# Autodesk Inventor assembly: L3 Gearbox Assembly
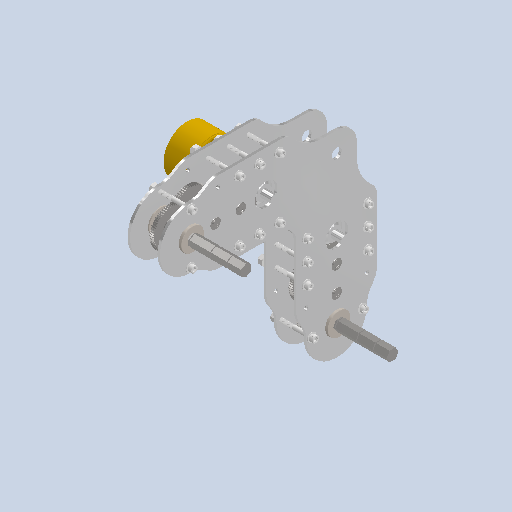
[picture p0: Inventor's stored thumbnail of the model, 512x512]
Saved by Autodesk Inventor 2025.1 (Build 291241020, 241B)
## iProperties
Created: 2023-02-14
Part Number: L3 Gearbox Assembly
Document SubType Name: Assembly
Designer: Dave
Mass: 1965.41 g
Surface Area: 3646.76 cm^2
Volume: 537.619 cm^3
Density: 3.65577 g/cm^3
Author: Dave
## Documents named in this file (16)
- C:\Users\t205b\OneDrive\Documents\Github\BehrendURCMechanical\CAD\Chassis V3\CH3-L3DoubleGearbox.iam
- C:\Users\t205b\OneDrive\Documents\Github\BehrendURCMechanical\CAD\Chassis V3\[Retired] GearBox\Final Gears and Assemblies\CH-1-01-20T_Drive Gear.ipt
- C:\Users\t205b\OneDrive\Documents\Github\BehrendURCMechanical\CAD\Chassis V3\[Retired] GearBox\Final Gears and Assemblies\CH-1-01-60T_Output.ipt
- C:\Users\t205b\OneDrive\Documents\Github\BehrendURCMechanical\CAD\Chassis V3\[Retired] GearBox\Final Gears and Assemblies\CH-1-01-20T_Idler.ipt
- C:\Users\t205b\OneDrive\Documents\Github\BehrendURCMechanical\CAD\Chassis V3\[Retired] GearBox\Final Gears and Assemblies\CH-1-01-60T_Idler.ipt
- C:\Users\t205b\OneDrive\Documents\Github\BehrendURCMechanical\CAD\Chassis V3\GearBox\Drive Motor Shaft Coupler.ipt
- C:\Users\t205b\OneDrive\Documents\Github\BehrendURCMechanical\CAD\Chassis V3\GearBox\Ch-1-01-0.5x4.5HexShaft.ipt
- C:\Users\t205b\OneDrive\Documents\Github\BehrendURCMechanical\CAD\Chassis V3\GearBox\CH-1-01-0.375x1.7TurnedHexShaft.ipt
- C:\Users\t205b\OneDrive\Documents\Github\BehrendURCMechanical\CAD\Chassis V3\GearBox\CH-1-01-0.5HexBearing.ipt
- C:\Users\t205b\OneDrive\Documents\Github\BehrendURCMechanical\CAD\Chassis V3\GearBox\CH-1-01-0.25IDSmoothBoreBearing.ipt
- C:\Users\t205b\OneDrive\Documents\Github\BehrendURCMechanical\CAD\Chassis V3\DriveMotorAssem\DriveMotorAssem.iam
- C:\Users\t205b\OneDrive\Documents\Github\BehrendURCMechanical\CAD\Chassis V3\Hardware\91251A252_Black-Oxide Alloy Steel Socket Head Screw.ipt
- C:\Users\t205b\OneDrive\Documents\Github\BehrendURCMechanical\CAD\Chassis V3\Hardware\91831A011_18-8 Stainless Steel Nylon-Insert Locknut.ipt
- C:\Users\t205b\OneDrive\Documents\Github\BehrendURCMechanical\CAD\Chassis V3\Hardware\90107A011_316 Stainless Steel Washer.ipt
- C:\Users\t205b\OneDrive\Documents\Github\BehrendURCMechanical\CAD\Chassis V3\L3Plate.ipt
- C:\Users\t205b\OneDrive\Documents\Github\BehrendURCMechanical\CAD\Chassis V3\CH-L3GearboxCover.ipt
## Components (100 placed, 15 different names)
1. L3Plate:1 — Insert:13, Insert:14, Insert:15, Insert:16, Insert:17, Insert:18, Insert:19, Insert:20, Flush:9, Mate:33, Mate:34, Mate:38, Mate:39
2. L3Plate:2 — Insert:39, Insert:41, Mate:35, Mate:37, Mate:41
3. CH-1-01-0.25IDSmoothBoreBearing:4 — Mate:10, Mate:21
4. CH-L3GearboxCover:1 — Mate:38, Mate:39, Mate:40, Mate:41
5. DriveMotorAssem:1 [sub-assembly] — Mate:27, Mate:30, Mate:37
6. 91831A011_18-8 Stainless Steel Nylon-Insert Locknut:4 — Insert:36
7. 91251A252_Black-Oxide Alloy Steel Socket Head Screw:1 — Insert:27
8. 90107A011_316 Stainless Steel Washer:1 — Insert:36
9. 91831A011_18-8 Stainless Steel Nylon-Insert Locknut:3 — Insert:37
10. 90107A011_316 Stainless Steel Washer:4 — Insert:37
11. 91251A252_Black-Oxide Alloy Steel Socket Head Screw:2 — Insert:28, Mate:40
12. 90107A011_316 Stainless Steel Washer:6 — Insert:38
13. 91251A252_Black-Oxide Alloy Steel Socket Head Screw:5 — Insert:30
14. 91831A011_18-8 Stainless Steel Nylon-Insert Locknut:2 — Insert:38
15. 91251A252_Black-Oxide Alloy Steel Socket Head Screw:6 — Insert:33
16. 91831A011_18-8 Stainless Steel Nylon-Insert Locknut:5 — Insert:42
17. 90107A011_316 Stainless Steel Washer:12 — Insert:42, Mate:35
18. 91251A252_Black-Oxide Alloy Steel Socket Head Screw:7 — Insert:34
19. 91831A011_18-8 Stainless Steel Nylon-Insert Locknut:6 — Insert:43
20. 90107A011_316 Stainless Steel Washer:14 — Insert:43
21. 91251A252_Black-Oxide Alloy Steel Socket Head Screw:8 — Insert:35
22. 91831A011_18-8 Stainless Steel Nylon-Insert Locknut:8 — Insert:44
23. 90107A011_316 Stainless Steel Washer:16 — Insert:44
24. 91251A252_Black-Oxide Alloy Steel Socket Head Screw:4 — Insert:32
25. 91831A011_18-8 Stainless Steel Nylon-Insert Locknut:7 — Insert:40
26. 90107A011_316 Stainless Steel Washer:10 — Insert:40, Insert:41
27. 91251A252_Black-Oxide Alloy Steel Socket Head Screw:3 — Insert:31
28. 91831A011_18-8 Stainless Steel Nylon-Insert Locknut:1 — Insert:45
29. 90107A011_316 Stainless Steel Washer:8 — Insert:39, Insert:45
30. CH-1-01-0.5HexBearing:1 — Mate:17, Flush:8
31. Ch-1-01-0.5x4.5HexShaft:1 — Mate:8, Mate:9, Flush:8
32. CH-1-01-0.25IDSmoothBoreBearing:3 — Mate:18, Mate:22, Mate:28, Mate:36
33. CH-1-01-0.375x1.7TurnedHexShaft:2 — Insert:12, Mate:28
34. Drive Motor Shaft Coupler:1 — Mate:27, Mate:30, Insert:29
35. CH-1-01-0.25IDSmoothBoreBearing:2 — Mate:32
36. CH-1-01-0.375x1.7TurnedHexShaft:1 — Mate:32, Flush:9
37. CH-1-01-0.25IDSmoothBoreBearing:1 — Insert:12, Mate:33
38. CH-1-01-0.5HexBearing:2 — Mate:8, Mate:9
39. CH-1-01-20T_Drive Gear:1 — Insert:29
40. CH-1-01-60T_Idler:2 — Mate:10, Mate:34
41. CH-1-01-20T_Idler:1 — Mate:21, Flush:5
42. CH-1-01-60T_Idler:1 — Mate:18, Mate:19, Flush:5, Mate:36
43. CH-1-01-20T_Idler:2 — Mate:19, Mate:22, Flush:6
44. CH-1-01-60T_Output:1 — Mate:17, Flush:6
45. 90107A011_316 Stainless Steel Washer:11 — Insert:18, Insert:33
46. 90107A011_316 Stainless Steel Washer:13 — Insert:19, Insert:34
47. 90107A011_316 Stainless Steel Washer:15 — Insert:20, Insert:35
48. 90107A011_316 Stainless Steel Washer:9 — Insert:17, Insert:32
49. 90107A011_316 Stainless Steel Washer:7 — Insert:16, Insert:31
50. 90107A011_316 Stainless Steel Washer:5 — Insert:15, Insert:30
51. 90107A011_316 Stainless Steel Washer:3 — Insert:14, Insert:28
52. 90107A011_316 Stainless Steel Washer:2 — Insert:13, Insert:27
53. DriveMotorAssem:2 [sub-assembly]
54. 91831A011_18-8 Stainless Steel Nylon-Insert Locknut:9
55. 91251A252_Black-Oxide Alloy Steel Socket Head Screw:9
56. 90107A011_316 Stainless Steel Washer:17
57. 91831A011_18-8 Stainless Steel Nylon-Insert Locknut:10
58. 90107A011_316 Stainless Steel Washer:18
59. 91251A252_Black-Oxide Alloy Steel Socket Head Screw:10
60. 90107A011_316 Stainless Steel Washer:19
61. 91251A252_Black-Oxide Alloy Steel Socket Head Screw:11
62. 91831A011_18-8 Stainless Steel Nylon-Insert Locknut:11
63. 91251A252_Black-Oxide Alloy Steel Socket Head Screw:12
64. 91831A011_18-8 Stainless Steel Nylon-Insert Locknut:12
65. 90107A011_316 Stainless Steel Washer:20
66. 91251A252_Black-Oxide Alloy Steel Socket Head Screw:13
67. 91831A011_18-8 Stainless Steel Nylon-Insert Locknut:13
68. 90107A011_316 Stainless Steel Washer:21
69. 91251A252_Black-Oxide Alloy Steel Socket Head Screw:14
70. 91831A011_18-8 Stainless Steel Nylon-Insert Locknut:14
71. 90107A011_316 Stainless Steel Washer:22
72. 91251A252_Black-Oxide Alloy Steel Socket Head Screw:15
73. 91831A011_18-8 Stainless Steel Nylon-Insert Locknut:15
74. 90107A011_316 Stainless Steel Washer:23
75. 91251A252_Black-Oxide Alloy Steel Socket Head Screw:16
76. 91831A011_18-8 Stainless Steel Nylon-Insert Locknut:16
77. 90107A011_316 Stainless Steel Washer:24
78. CH-1-01-0.5HexBearing:3
79. Ch-1-01-0.5x4.5HexShaft:2
80. CH-1-01-0.25IDSmoothBoreBearing:5
81. CH-1-01-0.375x1.7TurnedHexShaft:3
82. Drive Motor Shaft Coupler:2
83. CH-1-01-0.25IDSmoothBoreBearing:6
84. CH-1-01-0.375x1.7TurnedHexShaft:4
85. CH-1-01-0.25IDSmoothBoreBearing:7
86. CH-1-01-0.5HexBearing:4
87. CH-1-01-20T_Drive Gear:2
88. CH-1-01-60T_Idler:3
89. CH-1-01-20T_Idler:3
90. CH-1-01-60T_Idler:4
91. CH-1-01-20T_Idler:4
92. CH-1-01-60T_Output:2
93. 90107A011_316 Stainless Steel Washer:25
94. 90107A011_316 Stainless Steel Washer:26
95. 90107A011_316 Stainless Steel Washer:27
96. 90107A011_316 Stainless Steel Washer:28
97. 90107A011_316 Stainless Steel Washer:29
98. 90107A011_316 Stainless Steel Washer:30
99. 90107A011_316 Stainless Steel Washer:31
100. 90107A011_316 Stainless Steel Washer:32
## Component patterns: (2 elements, first: DriveMotorAssem:1 + 91831A011_18-8 Stainless Steel Nylon-Insert Locknut:4 + 91251A252_Black-Oxide Alloy Steel Socket Head Screw:1 + 90107A011_316 Stainless Steel Washer:1 + 91831A011_18-8 Stainless Steel Nylon-Insert Locknut:3 + 90107A011_316 Stainless Steel Washer:4 + 91251A252_Black-Oxide Alloy Steel Socket Head Screw:2 + 90107A011_316 Stainless Steel Washer:6 + 91251A252_Black-Oxide Alloy Steel Socket Head Screw:5 + 91831A011_18-8 Stainless Steel Nylon-Insert Locknut:2 + 91251A252_Black-Oxide Alloy Steel Socket Head Screw:6 + 91831A011_18-8 Stainless Steel Nylon-Insert Locknut:5 + 90107A011_316 Stainless Steel Washer:12 + 91251A252_Black-Oxide Alloy Steel Socket Head Screw:7 + 91831A011_18-8 Stainless Steel Nylon-Insert Locknut:6 + 90107A011_316 Stainless Steel Washer:14 + 91251A252_Black-Oxide Alloy Steel Socket Head Screw:8 + 91831A011_18-8 Stainless Steel Nylon-Insert Locknut:8 + 90107A011_316 Stainless Steel Washer:16 + 91251A252_Black-Oxide Alloy Steel Socket Head Screw:4 + 91831A011_18-8 Stainless Steel Nylon-Insert Locknut:7 + 90107A011_316 Stainless Steel Washer:10 + 91251A252_Black-Oxide Alloy Steel Socket Head Screw:3 + 91831A011_18-8 Stainless Steel Nylon-Insert Locknut:1 + 90107A011_316 Stainless Steel Washer:8 + CH-1-01-0.5HexBearing:1 + Ch-1-01-0.5x4.5HexShaft:1 + CH-1-01-0.25IDSmoothBoreBearing:3 + CH-1-01-0.375x1.7TurnedHexShaft:2 + Drive Motor Shaft Coupler:1 + CH-1-01-0.25IDSmoothBoreBearing:2 + CH-1-01-0.375x1.7TurnedHexShaft:1 + CH-1-01-0.25IDSmoothBoreBearing:1 + CH-1-01-0.5HexBearing:2 + CH-1-01-20T_Drive Gear:1 + CH-1-01-60T_Idler:2 + CH-1-01-20T_Idler:1 + CH-1-01-60T_Idler:1 + CH-1-01-20T_Idler:2 + CH-1-01-60T_Output:1 + 90107A011_316 Stainless Steel Washer:11 + 90107A011_316 Stainless Steel Washer:13 + 90107A011_316 Stainless Steel Washer:15 + 90107A011_316 Stainless Steel Washer:9 + 90107A011_316 Stainless Steel Washer:7 + 90107A011_316 Stainless Steel Washer:5 + 90107A011_316 Stainless Steel Washer:3 + 90107A011_316 Stainless Steel Washer:2)
## Relationships (62: Insert 34, Mate 22, Flush 5, Angle 1)
- [Angle] (0 deg): L3Plate:1
- [Flush]: L3Plate:1 ↔ L3Plate:2
- [Insert]: L3Plate:1 ↔ CH-1-01-0.25IDSmoothBoreBearing:1
- [Insert]: L3Plate:1 ↔ CH-1-01-0.25IDSmoothBoreBearing:2
- [Insert]: L3Plate:2 ↔ CH-1-01-0.25IDSmoothBoreBearing:3
- [Insert]: L3Plate:2 ↔ CH-1-01-0.25IDSmoothBoreBearing:4
- [Insert]: L3Plate:1 ↔ CH-1-01-0.5HexBearing:2
- [Insert]: L3Plate:2 ↔ CH-1-01-0.5HexBearing:1
- Mate:8: Ch-1-01-0.5x4.5HexShaft:1 ↔ CH-1-01-0.5HexBearing:2
- Mate:9: Ch-1-01-0.5x4.5HexShaft:1 ↔ CH-1-01-0.5HexBearing:2
- Insert:12: CH-1-01-0.375x1.7TurnedHexShaft:2 ↔ CH-1-01-0.25IDSmoothBoreBearing:1
- Mate:10: CH-1-01-0.25IDSmoothBoreBearing:4 ↔ CH-1-01-60T_Idler:2
- Mate:17: CH-1-01-0.5HexBearing:1 ↔ CH-1-01-60T_Output:1
- Mate:18: CH-1-01-0.25IDSmoothBoreBearing:3 ↔ CH-1-01-60T_Idler:1
- Mate:19: CH-1-01-60T_Idler:1 ↔ CH-1-01-20T_Idler:2
- Mate:21: CH-1-01-0.25IDSmoothBoreBearing:4 ↔ CH-1-01-20T_Idler:1
- Flush:5: CH-1-01-20T_Idler:1 ↔ CH-1-01-60T_Idler:1
- Mate:22: CH-1-01-0.25IDSmoothBoreBearing:3 ↔ CH-1-01-20T_Idler:2
- Flush:6: CH-1-01-20T_Idler:2 ↔ CH-1-01-60T_Output:1
- Flush:8: CH-1-01-0.5HexBearing:1 ↔ Ch-1-01-0.5x4.5HexShaft:1
- [Mate]: L3Plate:1 ↔ Drive Motor Shaft Coupler:1
- Mate:27: DriveMotorAssem:1 ↔ Drive Motor Shaft Coupler:1
- Mate:28: CH-1-01-0.25IDSmoothBoreBearing:3 ↔ CH-1-01-0.375x1.7TurnedHexShaft:2
- Insert:13: L3Plate:1 ↔ 90107A011_316 Stainless Steel Washer:2
- Insert:14: L3Plate:1 ↔ 90107A011_316 Stainless Steel Washer:3
- Insert:15: L3Plate:1 ↔ 90107A011_316 Stainless Steel Washer:5
- Insert:16: L3Plate:1 ↔ 90107A011_316 Stainless Steel Washer:7
- Insert:17: L3Plate:1 ↔ 90107A011_316 Stainless Steel Washer:9
- Insert:18: L3Plate:1 ↔ 90107A011_316 Stainless Steel Washer:11
- Insert:19: L3Plate:1 ↔ 90107A011_316 Stainless Steel Washer:13
- Insert:20: L3Plate:1 ↔ 90107A011_316 Stainless Steel Washer:15
- Insert:27: 91251A252_Black-Oxide Alloy Steel Socket Head Screw:1 ↔ 90107A011_316 Stainless Steel Washer:2
- Insert:28: 91251A252_Black-Oxide Alloy Steel Socket Head Screw:2 ↔ 90107A011_316 Stainless Steel Washer:3
- Mate:30: DriveMotorAssem:1 ↔ Drive Motor Shaft Coupler:1
- Insert:29: Drive Motor Shaft Coupler:1 ↔ CH-1-01-20T_Drive Gear:1
- Insert:30: 91251A252_Black-Oxide Alloy Steel Socket Head Screw:5 ↔ 90107A011_316 Stainless Steel Washer:5
- Insert:31: 91251A252_Black-Oxide Alloy Steel Socket Head Screw:3 ↔ 90107A011_316 Stainless Steel Washer:7
- Insert:32: 91251A252_Black-Oxide Alloy Steel Socket Head Screw:4 ↔ 90107A011_316 Stainless Steel Washer:9
- Insert:33: 91251A252_Black-Oxide Alloy Steel Socket Head Screw:6 ↔ 90107A011_316 Stainless Steel Washer:11
- Insert:34: 91251A252_Black-Oxide Alloy Steel Socket Head Screw:7 ↔ 90107A011_316 Stainless Steel Washer:13
- Insert:35: 91251A252_Black-Oxide Alloy Steel Socket Head Screw:8 ↔ 90107A011_316 Stainless Steel Washer:15
- Insert:36: 91831A011_18-8 Stainless Steel Nylon-Insert Locknut:4 ↔ 90107A011_316 Stainless Steel Washer:1
- Insert:37: 91831A011_18-8 Stainless Steel Nylon-Insert Locknut:3 ↔ 90107A011_316 Stainless Steel Washer:4
- Insert:38: 90107A011_316 Stainless Steel Washer:6 ↔ 91831A011_18-8 Stainless Steel Nylon-Insert Locknut:2
- Insert:39: L3Plate:2 ↔ 90107A011_316 Stainless Steel Washer:8
- Insert:40: 91831A011_18-8 Stainless Steel Nylon-Insert Locknut:7 ↔ 90107A011_316 Stainless Steel Washer:10
- Insert:41: L3Plate:2 ↔ 90107A011_316 Stainless Steel Washer:10
- Insert:42: 91831A011_18-8 Stainless Steel Nylon-Insert Locknut:5 ↔ 90107A011_316 Stainless Steel Washer:12
- Insert:43: 91831A011_18-8 Stainless Steel Nylon-Insert Locknut:6 ↔ 90107A011_316 Stainless Steel Washer:14
- Insert:44: 91831A011_18-8 Stainless Steel Nylon-Insert Locknut:8 ↔ 90107A011_316 Stainless Steel Washer:16
- Insert:45: 91831A011_18-8 Stainless Steel Nylon-Insert Locknut:1 ↔ 90107A011_316 Stainless Steel Washer:8
- Mate:32: CH-1-01-0.25IDSmoothBoreBearing:2 ↔ CH-1-01-0.375x1.7TurnedHexShaft:1
- Flush:9: L3Plate:1 ↔ CH-1-01-0.375x1.7TurnedHexShaft:1
- Mate:33: L3Plate:1 ↔ CH-1-01-0.25IDSmoothBoreBearing:1
- Mate:34: L3Plate:1 ↔ CH-1-01-60T_Idler:2
- Mate:35: L3Plate:2 ↔ 90107A011_316 Stainless Steel Washer:12
- Mate:36: CH-1-01-0.25IDSmoothBoreBearing:3 ↔ CH-1-01-60T_Idler:1
- Mate:37: L3Plate:2 ↔ DriveMotorAssem:1
- Mate:38: L3Plate:1 ↔ CH-L3GearboxCover:1
- Mate:39: L3Plate:1 ↔ CH-L3GearboxCover:1
- Mate:40: CH-L3GearboxCover:1 ↔ 91251A252_Black-Oxide Alloy Steel Socket Head Screw:2
- Mate:41: L3Plate:2 ↔ CH-L3GearboxCover:1
